# Autodesk Inventor assembly: other side of drivetrain
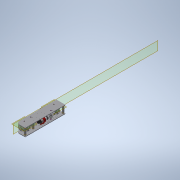
[picture p0: Inventor's stored thumbnail of the model, 180x180]
Saved by Autodesk Inventor 2020 (Build 240168000, 168)
## iProperties
Created: 2019-10-04
Part Number: other side of drivetrain
Document SubType Name: Assembly
Designer: ball
Author: ball
## Documents named in this file (10)
- D:\FTC8863\2019 Robot\Mecanum Drive Train\other side of drivetrain.iam
- D:\FTC8863\2019 Robot\Mecanum Drive Train\wheel with drive motor top_MIR.iam
- D:\FTC8863\2019 Robot\Mecanum Drive Train\wheel with drive motor floor_MIR.iam
- D:\FTC8863\2019 Robot\Mecanum Drive Train\inside wall_MIR.ipt
- D:\FTC8863\2019 Robot\Mecanum Drive Train\center motor mount_MIR.ipt
- D:\FTC8863\2019 Robot\Mecanum Drive Train\outside wall_MIR.ipt
- D:\FTC8863\2019 Robot\Mecanum Drive Train\motor mount cap_MIR.ipt
- D:\FTC8863\2019 Robot\Odoemetry module\OdometryAssembly_MIR.iam
- D:\FTC8863\2019 Robot\Mecanum Drive Train\odometry standoff_MIR.ipt
- D:\FTC8863\2019 Robot\Mecanum Drive Train\standoff for walls_MIR.ipt
## Components (12 placed, 9 different names)
1. wheel with drive motor top_MIR:1 [sub-assembly] — Flush:13, Mate:27, Flush:14, Mate:30, Mate:31, Mate:32, Mate:34
2. wheel with drive motor floor_MIR:1 [sub-assembly] — Flush:13, Mate:27, Flush:14, Mate:29, Mate:33
3. inside wall_MIR:1 — Mate:28, Mate:29, Mate:30, Mate:31, Angle:7, Mate:41, Mate:42, Angle:8, Mate:43, Mate:44
4. center motor mount_MIR:1 — Flush:15, Flush:16
5. outside wall_MIR:1 — Mate:32, Mate:33, Mate:34, Angle:5, Mate:35, Mate:36, Angle:6, Mate:39, Mate:40
6. motor mount cap_MIR:1 — Flush:15
7. motor mount cap_MIR:2 — Flush:16
8. OdometryAssembly_MIR:1 [sub-assembly] — Angle:5, Mate:35, Mate:36, Mate:37, Mate:38
9. odometry standoff_MIR:1 — Mate:37, Mate:38
10. standoff for walls_MIR:1 — Angle:6, Mate:39, Mate:40
11. standoff for walls_MIR:2 — Angle:7, Mate:41, Mate:42
12. standoff for walls_MIR:3 — Angle:8, Mate:43, Mate:44
## Relationships (26: Mate 18, Flush 4, Angle 4)
- Flush:13 (-330.2 mm): wheel with drive motor top_MIR:1 ↔ wheel with drive motor floor_MIR:1
- Mate:27 (44.3484 mm): wheel with drive motor top_MIR:1 ↔ wheel with drive motor floor_MIR:1
- Flush:14: wheel with drive motor top_MIR:1 ↔ wheel with drive motor floor_MIR:1
- Mate:28: inside wall_MIR:1
- Mate:29: wheel with drive motor floor_MIR:1 ↔ inside wall_MIR:1
- Mate:30: wheel with drive motor top_MIR:1 ↔ inside wall_MIR:1
- Mate:31: wheel with drive motor top_MIR:1 ↔ inside wall_MIR:1
- Mate:32: wheel with drive motor top_MIR:1 ↔ outside wall_MIR:1
- Mate:33: wheel with drive motor floor_MIR:1 ↔ outside wall_MIR:1
- Mate:34: wheel with drive motor top_MIR:1 ↔ outside wall_MIR:1
- Flush:15: center motor mount_MIR:1 ↔ motor mount cap_MIR:1
- Flush:16: center motor mount_MIR:1 ↔ motor mount cap_MIR:2
- Angle:5 (-10 deg): outside wall_MIR:1 ↔ OdometryAssembly_MIR:1
- Mate:35: outside wall_MIR:1 ↔ OdometryAssembly_MIR:1
- Mate:36 (1.27 mm): outside wall_MIR:1 ↔ OdometryAssembly_MIR:1
- Mate:37: OdometryAssembly_MIR:1 ↔ odometry standoff_MIR:1
- Mate:38: OdometryAssembly_MIR:1 ↔ odometry standoff_MIR:1
- Angle:6 (0 deg): outside wall_MIR:1 ↔ standoff for walls_MIR:1
- Mate:39: outside wall_MIR:1 ↔ standoff for walls_MIR:1
- Mate:40: outside wall_MIR:1 ↔ standoff for walls_MIR:1
- Angle:7 (0 deg): inside wall_MIR:1 ↔ standoff for walls_MIR:2
- Mate:41: inside wall_MIR:1 ↔ standoff for walls_MIR:2
- Mate:42: inside wall_MIR:1 ↔ standoff for walls_MIR:2
- Angle:8 (0 deg): inside wall_MIR:1 ↔ standoff for walls_MIR:3
- Mate:43: inside wall_MIR:1 ↔ standoff for walls_MIR:3
- Mate:44: inside wall_MIR:1 ↔ standoff for walls_MIR:3
